# Autodesk Inventor assembly: Test tube rack
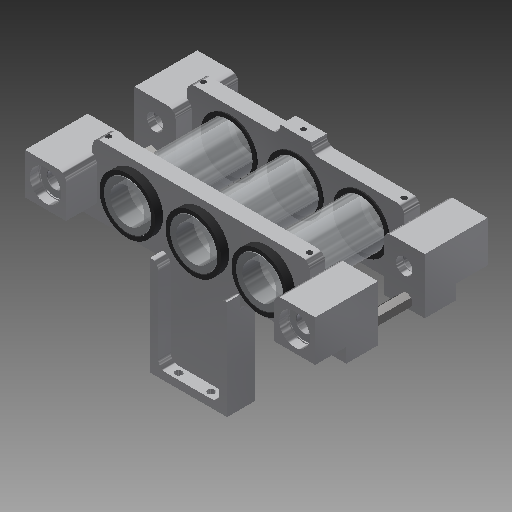
[picture p0: Inventor's stored thumbnail of the model, 512x512]
Saved by Autodesk Inventor 2017 (Build 210142000, 142)
## iProperties
Created: 2016-12-06
Part Number: Test tube rack
Document SubType Name: Assembly
Designer: qupec
Author: qupec
## Documents named in this file (10)
- C:\UMD\BPP\ROCKSAT X\star\CAD\Mechanical\Subsystems\Test Tube Rack\Test tube rack.iam
- C:\UMD\BPP\ROCKSAT X\star\CAD\Mechanical\Subsystems\Test Tube Rack\Test Tube.ipt
- C:\UMD\BPP\ROCKSAT X\star\CAD\Mechanical\Subsystems\Test Tube Rack\Tube Holder with camera attachment.ipt
- C:\UMD\BPP\ROCKSAT X\star\CAD\Mechanical\Subsystems\Test Tube Rack\Tube grip.ipt
- C:\UMD\BPP\ROCKSAT X\star\CAD\Mechanical\Subsystems\Test Tube Rack\Tube Holder Halve.ipt
- C:\UMD\BPP\ROCKSAT X\star\CAD\Mechanical\Subsystems\Test Tube Rack\Tube Holder Halve 2.ipt
- C:\UMD\BPP\ROCKSAT X\star\CAD\Mechanical\Subsystems\Test Tube Rack\Tube Holder Halve 3.ipt
- C:\Users\qupec\Documents\Inventor\Content Center Files\R2017\en-US\U UNC 2603(1)\Unbrako - 4 x 1 - 48 - 1 - Unbrako.ipt
- C:\UMD\BPP\ROCKSAT X\star\CAD\Mechanical\Subsystems\Test Tube Rack\LINEAR SLEEVE BRNG.ipt
- C:\UMD\BPP\ROCKSAT X\star\CAD\Mechanical\Spacer fot test tube rack.ipt
## Components (23 placed, 9 different names)
1. Tube Holder Halve:1 — Mate:10, Mate:11, Mate:46, Mate:53, Mate:57, Mate:59, Mate:61, Mate:62, Mate:65, Mate:67, Mate:69, Mate:71, Mate:72, Mate:74, Mate:75
2. Tube Holder Halve 2:1 — Mate:7, Mate:8, Mate:9, Mate:10, Mate:11, Mate:45, Mate:48, Mate:61
3. Tube grip:1 — Mate:3, Flush:6
4. Tube grip:2 — Mate:2, Flush:3
5. Tube grip:3 — Mate:4, Flush:5, Mate:8
6. Tube grip:4 — Mate:5, Flush:2, Mate:9
7. Tube grip:5 — Mate:1, Flush:4, Mate:7
8. Tube grip:6 — Mate:6, Flush:1
9. Test Tube:1 — Mate:5, Mate:6, Flush:1, Flush:2, Flush:13
10. Test Tube:2 — Mate:3, Mate:4, Flush:5, Flush:6, Flush:12
11. Test Tube:3 — Mate:1, Mate:2, Flush:3, Flush:4, Flush:11
12. Tube Holder with camera attachment:1 — Mate:26, Mate:27, Mate:55, Mate:56, Mate:58, Mate:60, Mate:63, Mate:64, Mate:66, Mate:68, Mate:70, Flush:14, Mate:73, Mate:76, Mate:77
13. Tube Holder Halve 3:1 — Mate:26, Mate:27, Flush:11, Flush:12, Flush:13, Mate:49, Mate:50, Mate:60
14. Unbrako UNC Hex Socket Cap - Inch 4 x 1 - Unbrako:1 — Mate:45, Mate:46, Mate:59
15. Unbrako UNC Hex Socket Cap - Inch 4 x 1 - Unbrako:2 — Mate:50, Mate:58
16. Unbrako UNC Hex Socket Cap - Inch 4 x 1 - Unbrako:3 — Mate:49, Mate:55, Mate:56
17. Unbrako UNC Hex Socket Cap - Inch 4 x 1 - Unbrako:4 — Mate:48, Mate:53, Mate:57
18. LINEAR SLEEVE BRNG:1 — Mate:63, Mate:68
19. LINEAR SLEEVE BRNG:2 — Mate:62, Mate:69
20. LINEAR SLEEVE BRNG:3 — Mate:65, Mate:67
21. LINEAR SLEEVE BRNG:4 — Mate:64, Mate:66
22. Spacer fot test tube rack:1 — Mate:74, Mate:75, Mate:76
23. Spacer fot test tube rack:2 — Mate:71, Mate:72, Mate:73, Mate:77
## Relationships (52: Mate 42, Flush 10)
- Mate:1: Tube grip:5 ↔ Test Tube:3
- Mate:2: Tube grip:2 ↔ Test Tube:3
- Mate:3: Tube grip:1 ↔ Test Tube:2
- Mate:4: Tube grip:3 ↔ Test Tube:2
- Mate:5: Tube grip:4 ↔ Test Tube:1
- Mate:6: Tube grip:6 ↔ Test Tube:1
- Flush:1: Tube grip:6 ↔ Test Tube:1
- Flush:2: Tube grip:4 ↔ Test Tube:1
- Flush:3: Tube grip:2 ↔ Test Tube:3
- Flush:4: Tube grip:5 ↔ Test Tube:3
- Flush:5: Tube grip:3 ↔ Test Tube:2
- Flush:6: Tube grip:1 ↔ Test Tube:2
- Mate:7: Tube Holder Halve 2:1 ↔ Tube grip:5
- Mate:8: Tube Holder Halve 2:1 ↔ Tube grip:3
- Mate:9: Tube Holder Halve 2:1 ↔ Tube grip:4
- Mate:10: Tube Holder Halve:1 ↔ Tube Holder Halve 2:1
- Mate:11: Tube Holder Halve:1 ↔ Tube Holder Halve 2:1
- Mate:26: Tube Holder with camera attachment:1 ↔ Tube Holder Halve 3:1
- Mate:27: Tube Holder with camera attachment:1 ↔ Tube Holder Halve 3:1
- Flush:11 (-3.175 mm): Test Tube:3 ↔ Tube Holder Halve 3:1
- Flush:12 (-3.175 mm): Test Tube:2 ↔ Tube Holder Halve 3:1
- Flush:13 (-3.175 mm): Test Tube:1 ↔ Tube Holder Halve 3:1
- Mate:45: Tube Holder Halve 2:1 ↔ Unbrako UNC Hex Socket Cap - Inch 4 x 1 - Unbrako:1
- Mate:46: Tube Holder Halve:1 ↔ Unbrako UNC Hex Socket Cap - Inch 4 x 1 - Unbrako:1
- Mate:48: Tube Holder Halve 2:1 ↔ Unbrako UNC Hex Socket Cap - Inch 4 x 1 - Unbrako:4
- Mate:49: Tube Holder Halve 3:1 ↔ Unbrako UNC Hex Socket Cap - Inch 4 x 1 - Unbrako:3
- Mate:50: Tube Holder Halve 3:1 ↔ Unbrako UNC Hex Socket Cap - Inch 4 x 1 - Unbrako:2
- Mate:53: Tube Holder Halve:1 ↔ Unbrako UNC Hex Socket Cap - Inch 4 x 1 - Unbrako:4
- Mate:55: Tube Holder with camera attachment:1 ↔ Unbrako UNC Hex Socket Cap - Inch 4 x 1 - Unbrako:3
- Mate:56: Tube Holder with camera attachment:1 ↔ Unbrako UNC Hex Socket Cap - Inch 4 x 1 - Unbrako:3
- Mate:57: Tube Holder Halve:1 ↔ Unbrako UNC Hex Socket Cap - Inch 4 x 1 - Unbrako:4
- Mate:58: Tube Holder with camera attachment:1 ↔ Unbrako UNC Hex Socket Cap - Inch 4 x 1 - Unbrako:2
- Mate:59: Tube Holder Halve:1 ↔ Unbrako UNC Hex Socket Cap - Inch 4 x 1 - Unbrako:1
- Mate:60: Tube Holder with camera attachment:1 ↔ Tube Holder Halve 3:1
- Mate:61: Tube Holder Halve:1 ↔ Tube Holder Halve 2:1
- Mate:62: Tube Holder Halve:1 ↔ LINEAR SLEEVE BRNG:2
- Mate:63: Tube Holder with camera attachment:1 ↔ LINEAR SLEEVE BRNG:1
- Mate:64: Tube Holder with camera attachment:1 ↔ LINEAR SLEEVE BRNG:4
- Mate:65: Tube Holder Halve:1 ↔ LINEAR SLEEVE BRNG:3
- Mate:66: Tube Holder with camera attachment:1 ↔ LINEAR SLEEVE BRNG:4
- Mate:67: Tube Holder Halve:1 ↔ LINEAR SLEEVE BRNG:3
- Mate:68: Tube Holder with camera attachment:1 ↔ LINEAR SLEEVE BRNG:1
- Mate:69: Tube Holder Halve:1 ↔ LINEAR SLEEVE BRNG:2
- Mate:70: Tube Holder with camera attachment:1
- Flush:14: Tube Holder with camera attachment:1
- Mate:71: Tube Holder Halve:1 ↔ Spacer fot test tube rack:2
- Mate:72: Tube Holder Halve:1 ↔ Spacer fot test tube rack:2
- Mate:73: Tube Holder with camera attachment:1 ↔ Spacer fot test tube rack:2
- Mate:74: Tube Holder Halve:1 ↔ Spacer fot test tube rack:1
- Mate:75: Tube Holder Halve:1 ↔ Spacer fot test tube rack:1
- Mate:76: Tube Holder with camera attachment:1 ↔ Spacer fot test tube rack:1
- Mate:77: Tube Holder with camera attachment:1 ↔ Spacer fot test tube rack:2
